# Autodesk Inventor assembly: chain
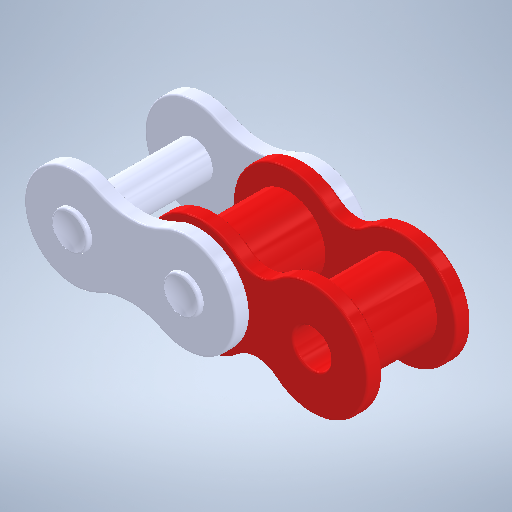
[picture p0: Inventor's stored thumbnail of the model, 512x512]
Saved by Autodesk Inventor 2026.1 (Build 301233020, 233B)
## iProperties
Created: 2026-01-22
Part Number: chain
Document SubType Name: Assembly
Designer: user
Author: user
## Documents named in this file (3)
- D:\asu\machine element design\project\design\chain.iam
- C:\Users\user\Downloads\chain-and-sporket-wheel-1.snapshot.1\1 outer chain\1 outer chain\1 outer chain.ipt
- C:\Users\user\Downloads\chain-and-sporket-wheel-1.snapshot.1\2 inner chain\2 inner chain\2 inner chain.ipt
## Components (2 placed, 2 different names)
1. 1 outer chain:1 — Mate:1, Mate:2
2. 2 inner chain:1 — Mate:1, Mate:2
## Relationships (2: Mate 2)
- Mate:1: 1 outer chain:1 ↔ 2 inner chain:1
- Mate:2: 1 outer chain:1 ↔ 2 inner chain:1
